# Autodesk Inventor assembly: SteelWaterTank
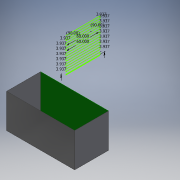
[picture p0: Inventor's stored thumbnail of the model, 180x180]
Saved by Autodesk Inventor 2019 (Build 230136000, 136)
## iProperties
Created: 2021-05-18
Part Number: SteelWaterTank
Document SubType Name: Weldment
Designer: jamieson-bl
Weld Material: Steel, Mild, Welded
Author: jamieson-bl
## Documents named in this file (3)
- \\Mac\Home\Desktop\DarkPoolDrawings\SteelWaterTank.iam
- \\Mac\Home\Desktop\DarkPoolDrawings\SteelTankSideandBottom.ipt
- \\Mac\Home\Desktop\DarkPoolDrawings\SteelTankEnds.ipt
## Components (5 placed, 2 different names)
1. SteelTankSideandBottom:1 — Flush:1, Mate:1, Flush:2, Mate:3, Mate:9
2. SteelTankSideandBottom:2 — Mate:4, Flush:4, Mate:5, Mate:7
3. SteelTankSideandBottom:3 — Flush:1, Mate:1, Flush:2, Mate:2, Flush:3, Mate:5, Mate:6, Flush:5, Mate:8
4. SteelTankEnds:1 — Mate:6, Flush:5, Mate:7, Mate:10
5. SteelTankEnds:2 — Mate:2, Mate:3, Flush:3, Mate:4, Flush:4
## Relationships (15: Mate 10, Flush 5)
- Flush:1: SteelTankSideandBottom:1 ↔ SteelTankSideandBottom:3
- Mate:1: SteelTankSideandBottom:1 ↔ SteelTankSideandBottom:3
- Flush:2: SteelTankSideandBottom:1 ↔ SteelTankSideandBottom:3
- Mate:2: SteelTankSideandBottom:3 ↔ SteelTankEnds:2
- Mate:3: SteelTankSideandBottom:1 ↔ SteelTankEnds:2
- Flush:3: SteelTankSideandBottom:3 ↔ SteelTankEnds:2
- Mate:4: SteelTankSideandBottom:2 ↔ SteelTankEnds:2
- Flush:4: SteelTankSideandBottom:2 ↔ SteelTankEnds:2
- Mate:5: SteelTankSideandBottom:2 ↔ SteelTankSideandBottom:3
- Mate:6: SteelTankSideandBottom:3 ↔ SteelTankEnds:1
- Flush:5: SteelTankSideandBottom:3 ↔ SteelTankEnds:1
- Mate:7: SteelTankSideandBottom:2 ↔ SteelTankEnds:1
- Mate:8: SteelTankSideandBottom:3
- Mate:9: SteelTankSideandBottom:1
- Mate:10: SteelTankEnds:1
## Named parameters: sa_0 = 980.999
note: some values were not read from the file. Shown as the stored number, unit unknown: "sa_0".
